# Autodesk Inventor assembly: Clamex P-10 Connector
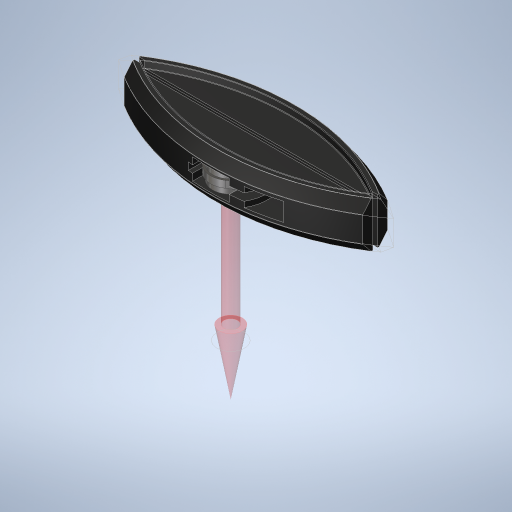
[picture p0: Inventor's stored thumbnail of the model, 512x512]
Saved by Autodesk Inventor 2024 (Build 280153000, 153)
## iProperties
Created: 2024-02-21
Part Number: Clamex P-10 Connector
Document SubType Name: Assembly
Designer: S. Dereškevičius
Author: S. Dereškevičius
## Documents named in this file (5)
- C:\W4INV 2024 Design\LIBRARY\Fixed joints\Lamello Clamex P-10\Clamex P-10 Connector.iam
- C:\W4INV 2024 Design\LIBRARY\Fixed joints\Lamello Clamex P-10\Clamex-P-10.ipt
- C:\W4INV 2024 Design\LIBRARY\Fixed joints\Lamello Clamex P-10\P-10-Nut_groove.ipt
- C:\W4INV 2024 Design\LIBRARY\Fixed joints\Lamello Clamex P-10\P-10-Nut_groove Without Drill.ipt
- C:\W4INV 2024 Design\LIBRARY\Fixed joints\Lamello Clamex P-14\Hole Direction Indicator.ipt
## Components (4 placed, 4 different names)
1. Clamex-P-10:1 — Mate:2, Flush:2, Mate:4, Insert:1, Angle:1, Insert:2, Angle:2, Insert:3
2. P-10-Nut_groove:1 — Insert:2, Angle:2
3. P-10-Nut_groove Without Drill:1 — Insert:1, Angle:1
4. Hole Direction Indicator:1 — Insert:3
## Relationships (8: Insert 3, Mate 2, Angle 2, Flush 1)
- Mate:2: Clamex-P-10:1
- Flush:2: Clamex-P-10:1
- Mate:4: Clamex-P-10:1
- Insert:1: Clamex-P-10:1 ↔ P-10-Nut_groove Without Drill:1
- Angle:1 (0 deg): Clamex-P-10:1 ↔ P-10-Nut_groove Without Drill:1
- Insert:2: Clamex-P-10:1 ↔ P-10-Nut_groove:1
- Angle:2 (0 deg): Clamex-P-10:1 ↔ P-10-Nut_groove:1
- Insert:3: Clamex-P-10:1 ↔ Hole Direction Indicator:1
